# Autodesk Inventor assembly: COXA_ROLL_LINK_ASM
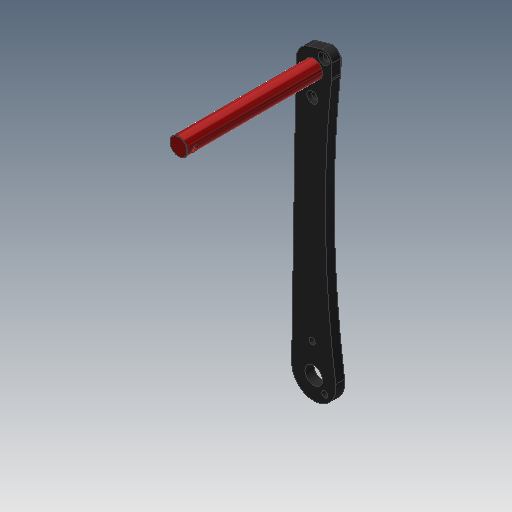
[picture p0: Inventor's stored thumbnail of the model, 512x512]
Saved by Autodesk Inventor 2019.4 (Build 234330000, 330)
## iProperties
Created: 2019-11-06
Part Number: COXA_ROLL_LINK_ASM
Material: 一般
Document SubType Name: Assembly
Designer: y6tada
Author: y6tada
## Documents named in this file (3)
- C:\Workspace\Yuni9\Inventor\Asm\COXA_UNIT\COXA_ROLL_LINK_ASM.iam
- C:\Workspace\Yuni9\Inventor\Asm\COXA_UNIT\COXA_ROLL_LONG-LINK.ipt
- C:\Workspace\Yuni9\Inventor\Asm\COXA_UNIT\COXA_ROLL_SHAFT_D4.ipt
## Components (2 placed, 2 different names)
1. COXA_ROLL_LONG-LINK:1 — フラッシュ:1, フラッシュ:2, フラッシュ:3, メイト:1
2. COXA_ROLL_SHAFT_D4:1 — メイト:1
## Relationships (4: Flush 3, Mate 1)
- フラッシュ:1 [Flush]: COXA_ROLL_LONG-LINK:1
- フラッシュ:2 [Flush]: COXA_ROLL_LONG-LINK:1
- フラッシュ:3 [Flush]: COXA_ROLL_LONG-LINK:1
- メイト:1 [Mate]: COXA_ROLL_LONG-LINK:1 ↔ COXA_ROLL_SHAFT_D4:1
